# Autodesk Inventor assembly: A135
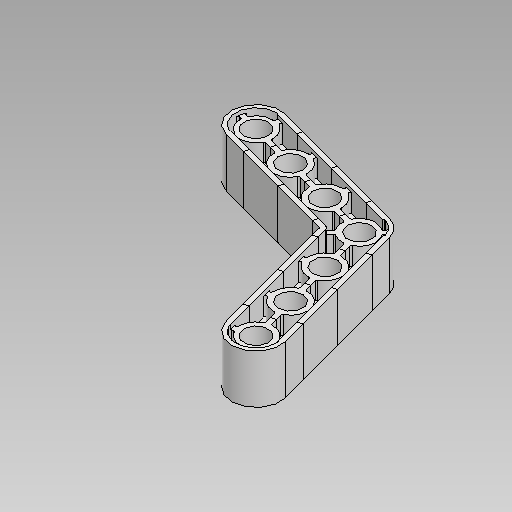
[picture p0: Inventor's stored thumbnail of the model, 512x512]
Saved by Autodesk Inventor 2020 (Build 240168000, 168)
## iProperties
Created: 2019-05-05
Part Number: A135
Document SubType Name: Assembly
Designer: Varga Daniel
Author: Varga Daniel
## Documents named in this file (5)
- C:\!_Dani\!_cloud\OneDrive\!_munka\Revolution\StructuralParts\Beams\Angled Beams\A120.iam
- C:\!_Dani\!_cloud\OneDrive\!_munka\Revolution\StructuralParts\Beams\Beam_bent_base.ipt
- C:\!_Dani\!_cloud\OneDrive\!_munka\Revolution\StructuralParts\Beams\beam_single_end_part.ipt
- C:\!_Dani\!_cloud\OneDrive\!_munka\Revolution\StructuralParts\Beams\beam_single_inner_part.ipt
- C:\!_Dani\!_cloud\OneDrive\!_munka\Revolution\StructuralParts\Beams\Beam_bent_base\Beam_bent_base-120.ipt
## Components (7 placed, 3 different names)
1. Beam_bent_base-120:1 — Mate:5, Flush:9, Flush:10, Flush:11, Flush:12, Mate:6
2. beam_single_end_part:1 — Flush:1, Flush:2, Mate:1
3. beam_single_inner_part:1 — Mate:2, Flush:3, Flush:4, Flush:11, Mate:6
4. beam_single_inner_part:2 — Flush:1, Flush:2, Mate:1, Mate:2, Flush:3, Flush:4, Flush:12
5. beam_single_end_part:2
6. beam_single_inner_part:3 — Mate:5, Flush:9, Flush:10
7. beam_single_inner_part:4
## Relationships (18: Flush 12, Mate 6)
- Flush:1: beam_single_end_part:1 ↔ beam_single_inner_part:2
- Flush:2: beam_single_end_part:1 ↔ beam_single_inner_part:2
- Mate:1: beam_single_end_part:1 ↔ beam_single_inner_part:2
- Mate:2: beam_single_inner_part:1 ↔ beam_single_inner_part:2
- Flush:3: beam_single_inner_part:1 ↔ beam_single_inner_part:2
- Flush:4: beam_single_inner_part:1 ↔ beam_single_inner_part:2
- [Flush]: beam_single_end_part:2 ↔ beam_single_inner_part:4
- [Flush]: beam_single_end_part:2 ↔ beam_single_inner_part:4
- [Mate]: beam_single_end_part:2 ↔ beam_single_inner_part:4
- [Mate]: beam_single_inner_part:3 ↔ beam_single_inner_part:4
- [Flush]: beam_single_inner_part:3 ↔ beam_single_inner_part:4
- [Flush]: beam_single_inner_part:3 ↔ beam_single_inner_part:4
- Mate:5: Beam_bent_base-120:1 ↔ beam_single_inner_part:3
- Flush:9: Beam_bent_base-120:1 ↔ beam_single_inner_part:3
- Flush:10: Beam_bent_base-120:1 ↔ beam_single_inner_part:3
- Flush:11: Beam_bent_base-120:1 ↔ beam_single_inner_part:1
- Flush:12: Beam_bent_base-120:1 ↔ beam_single_inner_part:2
- Mate:6: Beam_bent_base-120:1 ↔ beam_single_inner_part:1
## Named parameters: d6_d3 = 0 mm, d7_d4 = 0 mm, d8_d5 = 0 mm, d9_d0 = 0 mm, d10_d1 = 0 mm, d11_d2 = 0 mm
